# Autodesk Inventor assembly: battery_block_multipart_bigtouch
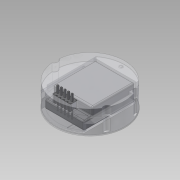
[picture p0: Inventor's stored thumbnail of the model, 180x180]
Saved by Autodesk Inventor 2015 SP2 (Build 190223200, 223)
## iProperties
Created: 2015-03-07
Part Number: battery_block_multipart_bigtouch
Document SubType Name: Assembly
Designer: Mathieu
Mass: 3.74293 g
Surface Area: 41.296 cm^2
Volume: 3.37428 cm^3
Density: 1.10925 g/cm^3
Author: Mathieu
## Documents named in this file (5)
- D:\Users\Mathieu\Desktop\SmartTokens\SmartTokens\Inventor Files\battery_block.iam
- D:\Users\Mathieu\Desktop\SmartTokens\SmartTokens\Inventor Files\battery.ipt
- D:\Users\Mathieu\Desktop\SmartTokens\SmartTokens\Inventor Files\bottom2_2.ipt
- D:\Users\Mathieu\Desktop\SmartTokens\SmartTokens\Inventor Files\bottom1_2.ipt
- D:\Users\Mathieu\Desktop\SmartTokens\SmartTokens\Inventor Files\battery_connector.ipt
## Components (4 placed, 4 different names)
1. battery:1 — Mate:11, Mate:12, Mate:13
2. bottom2_2:1 — Mate:14, Mate:16, Flush:1, Mate:17, Mate:18
3. bottom1_2:1 — Mate:11, Mate:12, Mate:13, Mate:14, Mate:16
4. battery_connector:1 — Flush:1, Mate:17, Mate:18
## Relationships (8: Mate 7, Flush 1)
- Mate:11 (0.25 mm): battery:1 ↔ bottom1_2:1
- Mate:12 (0.5 mm): battery:1 ↔ bottom1_2:1
- Mate:13: battery:1 ↔ bottom1_2:1
- Mate:14 (0.1 mm): bottom2_2:1 ↔ bottom1_2:1
- Mate:16 (0.1 mm): bottom2_2:1 ↔ bottom1_2:1
- Flush:1: bottom2_2:1 ↔ battery_connector:1
- Mate:17 (0.075 mm): bottom2_2:1 ↔ battery_connector:1
- Mate:18 (0.075 mm): bottom2_2:1 ↔ battery_connector:1
